# Autodesk Inventor assembly: B Drive
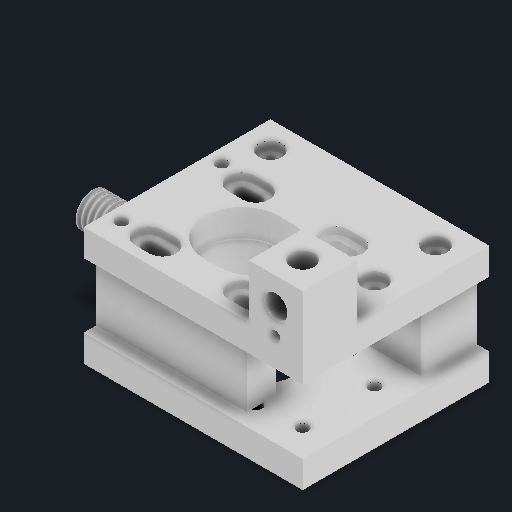
[picture p0: Inventor's stored thumbnail of the model, 512x512]
Saved by Autodesk Inventor 2025.1 (Build 291241020, 241B)
## iProperties
Created: 2025-04-19
Part Number: B Drive
Document SubType Name: Assembly
Designer: Joshua Eah
Author: Joshua Eah
## Documents named in this file (5)
- C:\Users\Joshua Eah\Documents\VORON 0.2 MACHINED PARTS\AB Drives\B Drive\B Drive.iam
- C:\Users\Joshua Eah\Documents\VORON 0.2 MACHINED PARTS\AB Drives\B Drive\B Drive Frame Lower.ipt
- C:\Users\Joshua Eah\Documents\VORON 0.2 MACHINED PARTS\AB Drives\B Drive\B Drive Frame Upper.ipt
- C:\Users\Joshua Eah\Documents\VORON 0.2 MACHINED PARTS\AB Drives\B Drive\B Drive Tensioner.ipt
- C:\Users\Joshua Eah\Documents\VORON 0.2 MACHINED PARTS\AB Drives\Drive Tensioner Rod\Tensioner Rod.ipt
## Components (4 placed, 4 different names)
1. B Drive Frame Lower:1 — Rigid:1, Cylindrical:1
2. B Drive Frame Upper:1 — Rigid:1
3. B Drive Tensioner:1 — Cylindrical:1, Rotational:1
4. Tensioner Rod:1 — Rotational:1
## Relationships (3: WeldJoint 1, CylindricalJoint 1, RevoluteJoint 1)
- Rigid:1 [WeldJoint]: B Drive Frame Lower:1 ↔ B Drive Frame Upper:1
- Cylindrical:1: B Drive Frame Lower:1 ↔ B Drive Tensioner:1
- Rotational:1 [RevoluteJoint]: B Drive Tensioner:1 ↔ Tensioner Rod:1
## Named parameters: Finish1_Area = 296.504
note: some values were not read from the file. Shown as the stored number, unit unknown: "Finish1_Area".
